# Autodesk Inventor assembly: Track Frame Assembly
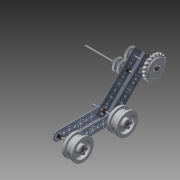
[picture p0: Inventor's stored thumbnail of the model, 180x180]
Saved by Autodesk Inventor 2015 (Build 190159000, 159)
## iProperties
Created: 2015-09-27
Part Number: Track Frame Assembly
Document SubType Name: Assembly
Designer: Jing-Chen
Author: Jing-Chen
## Documents named in this file (17)
- C:\Users\Jing-Chen\Desktop\Bionic Hybrids 2016\Bionic-Hybrids\CAD\Drivetrain\Sub-Assemblies\Track Frame Assembly.iam
- C:\Users\Jing-Chen\Desktop\Bionic Hybrids 2016\Bionic-Hybrids\Stock\Bracket-U9 - 739067.ipt
- C:\Users\Jing-Chen\Desktop\Bionic Hybrids 2016\Bionic-Hybrids\CAD\Drivetrain\Sub-Assemblies\Track Idler Assembly.iam
- C:\Users\Jing-Chen\Desktop\Bionic Hybrids 2016\Bionic-Hybrids\Stock\Bearing-Thrust - 739091.ipt
- C:\Users\Jing-Chen\Desktop\Bionic Hybrids 2016\Bionic-Hybrids\Stock\Shaft Collar-Setscrew, Axle - 739092.iam
- C:\Users\Jing-Chen\Desktop\Bionic Hybrids 2016\Bionic-Hybrids\Stock\Track Sprocket - 736468.ipt
- C:\Users\Jing-Chen\Desktop\Bionic Hybrids 2016\Bionic-Hybrids\Stock\Shaft Collar-Setscrew, Axle, Mountable - 739172.iam
- C:\Users\Jing-Chen\Desktop\Bionic Hybrids 2016\Bionic-Hybrids\Stock\Plate-9x1 - 739272.ipt
- C:\Users\Jing-Chen\Desktop\Bionic Hybrids 2016\Bionic-Hybrids\Stock\Spacer 3.125mm- 739100.ipt
- C:\Users\Jing-Chen\Desktop\Bionic Hybrids 2016\Bionic-Hybrids\Stock\Gear-40 tooth - 731901.ipt
- C:\Users\Jing-Chen\Desktop\Bionic Hybrids 2016\Bionic-Hybrids\Stock\Plate-1x1 - 739387.ipt
- C:\Users\Jing-Chen\Desktop\Bionic Hybrids 2016\Bionic-Hybrids\Stock\Screw 0.5in - 739097.ipt
- C:\Users\Jing-Chen\Desktop\Bionic Hybrids 2016\Bionic-Hybrids\CAD\General\Modified Parts\Cut 100mm axle.ipt
- C:\Users\Jing-Chen\Desktop\Bionic Hybrids 2016\Bionic-Hybrids\CAD\Drivetrain\Sub-Assemblies\Tread Sprocket Assembly.iam
- C:\Users\Jing-Chen\Desktop\Bionic Hybrids 2016\Bionic-Hybrids\Stock\Axle-250mm - 735871.ipt
- C:\Users\Jing-Chen\Desktop\Bionic Hybrids 2016\Bionic-Hybrids\CAD\General\Modified Parts\Axle Hub - non-locking.ipt
- C:\Users\Jing-Chen\Desktop\Bionic Hybrids 2016\Bionic-Hybrids\Stock\Axle-100mm - 739088.ipt
## Components (42 placed, 16 different names)
1. Bracket-U9 - 739067:1 — Mate:16, Mate:17, Mate:18, Mate:19, Mate:20, Mate:21, Mate:44, Mate:46, Mate:60, Mate:61, Mate:63, Mate:66, Mate:67, Mate:88, Mate:89, Mate:90, Mate:91, Mate:108, Mate:122, Mate:159, Mate:160, Mate:161, Mate:162, Mate:164, Mate:166, Mate:165, Mate:163
2. Track Idler Assembly:1 [sub-assembly] — Mate:43, Flush:9, Mate:134
3. Shaft Collar-Setscrew, Axle - 739092:1 [sub-assembly] — Mate:42, Mate:133
4. Track Sprocket - 736468:1 — Mate:13, Mate:15, Mate:105, Mate:126, Mate:135, Mate:136, Mate:137, Mate:138, Mate:139, Mate:140, Mate:141, Mate:142
5. Shaft Collar-Setscrew, Axle, Mountable - 739172:1 [sub-assembly] — Mate:13, Mate:15, Mate:22, Mate:105, Mate:106, Angle:3, Mate:109, Angle:5
6. Plate-9x1 - 739272:1 — Mate:16, Mate:19, Mate:21, Mate:37, Mate:38, Mate:45, Flush:4, Flush:5, Mate:53
7. Plate-9x1 - 739272:2 — Mate:17, Mate:18, Mate:20, Mate:39, Mate:40, Mate:47, Mate:179
8. Cut 100mm axle:1 — Mate:22, Mate:58, Mate:99, Mate:100, Mate:101, Angle:2, Angle:3, Mate:107, Angle:4, Mate:109, Angle:5, Mate:121, Mate:124, Mate:125, Flush:7
9. Bearing-Thrust - 739091:5 — Mate:44, Mate:45, Mate:50, Mate:175
10. Bearing-Thrust - 739091:6 — Mate:39, Mate:40, Mate:42, Mate:132
11. Bearing-Thrust - 739091:10 — Mate:46, Mate:47
12. Bearing-Thrust - 739091:11 — Mate:37, Mate:38, Mate:43
13. Track Idler Assembly:2 [sub-assembly] — Mate:50, Mate:176, Flush:10
14. Shaft Collar-Setscrew, Axle - 739092:2 [sub-assembly] — Mate:180, Mate:181
15. Gear-40 tooth - 731901:1 — Mate:55, Mate:57, Mate:64, Mate:84, Mate:85, Mate:86, Mate:87, Rotation:1
16. Shaft Collar-Setscrew, Axle, Mountable - 739172:2 [sub-assembly] — Mate:55, Mate:57, Mate:58, Mate:63, Mate:64, Angle:2, Mate:107, Mate:108, Angle:4
17. Shaft Collar-Setscrew, Axle, Mountable - 739172:4 [sub-assembly] — Mate:60, Mate:61, Mate:66, Angle:1
18. Axle-250mm - 735871:1 — Angle:1
19. Plate-1x1 - 739387:1 — Mate:67, Mate:70
20. Bearing-Thrust - 739091:12 — Mate:70, Mate:72
21. Spacer 3.125mm- 739100:3 — Mate:72, Mate:128
22. Screw 0.5in - 739097:1 — Mate:84, Mate:86
23. Screw 0.5in - 739097:2 — Mate:85, Mate:87
24. Screw 0.5in - 739097:3 — Mate:88, Mate:90
25. Screw 0.5in - 739097:4 — Mate:89, Mate:91
26. Spacer 3.125mm- 739100:5 — Mate:101, Mate:102, Mate:123, Mate:124
27. Spacer 3.125mm- 739100:6 — Mate:100, Mate:102, Mate:103
28. Spacer 3.125mm- 739100:7 — Mate:99, Mate:103, Mate:106
29. Bearing-Thrust - 739091:13 — Mate:121, Mate:122, Mate:123
30. Bearing-Thrust - 739091:14 — Mate:125, Mate:126, Flush:7
31. Tread Sprocket Assembly:1 [sub-assembly] — Mate:128, Rotation:1
32. Cut 100mm axle:3 — Flush:9, Mate:132, Mate:133, Mate:134
33. Screw 0.5in - 739097:5 — Mate:135, Mate:139
34. Screw 0.5in - 739097:6 — Mate:136, Mate:140
35. Screw 0.5in - 739097:7 — Mate:137, Mate:142
36. Screw 0.5in - 739097:8 — Mate:138, Mate:141
37. Screw 0.5in - 739097:13 — Mate:159, Mate:164, Mate:178
38. Screw 0.5in - 739097:14 — Mate:160, Mate:163
39. Screw 0.5in - 739097:15 — Mate:161, Mate:165
40. Screw 0.5in - 739097:16 — Mate:162, Mate:166
41. Axle Hub - non-locking:1 — Mate:177, Mate:178, Mate:179, Mate:181
42. Axle-100mm - 739088:1 — Mate:175, Mate:176, Flush:10, Mate:177, Mate:180
## Relationships (100: Mate 88, Flush 6, Angle 5, RelateRotation 1)
- Mate:13: Track Sprocket - 736468:1 ↔ Shaft Collar-Setscrew, Axle, Mountable - 739172:1
- Mate:15: Track Sprocket - 736468:1 ↔ Shaft Collar-Setscrew, Axle, Mountable - 739172:1
- Mate:16: Bracket-U9 - 739067:1 ↔ Plate-9x1 - 739272:1
- Mate:17: Bracket-U9 - 739067:1 ↔ Plate-9x1 - 739272:2
- Mate:18: Bracket-U9 - 739067:1 ↔ Plate-9x1 - 739272:2
- Mate:19: Bracket-U9 - 739067:1 ↔ Plate-9x1 - 739272:1
- Mate:20: Bracket-U9 - 739067:1 ↔ Plate-9x1 - 739272:2
- Mate:21: Bracket-U9 - 739067:1 ↔ Plate-9x1 - 739272:1
- Mate:22: Shaft Collar-Setscrew, Axle, Mountable - 739172:1 ↔ Cut 100mm axle:1
- Mate:37: Plate-9x1 - 739272:1 ↔ Bearing-Thrust - 739091:11
- Mate:38: Plate-9x1 - 739272:1 ↔ Bearing-Thrust - 739091:11
- Mate:39: Plate-9x1 - 739272:2 ↔ Bearing-Thrust - 739091:6
- Mate:40: Plate-9x1 - 739272:2 ↔ Bearing-Thrust - 739091:6
- Mate:42: Shaft Collar-Setscrew, Axle - 739092:1 ↔ Bearing-Thrust - 739091:6
- Mate:43: Track Idler Assembly:1 ↔ Bearing-Thrust - 739091:11
- Mate:44: Bracket-U9 - 739067:1 ↔ Bearing-Thrust - 739091:5
- Mate:45: Plate-9x1 - 739272:1 ↔ Bearing-Thrust - 739091:5
- Mate:46: Bracket-U9 - 739067:1 ↔ Bearing-Thrust - 739091:10
- Mate:47: Plate-9x1 - 739272:2 ↔ Bearing-Thrust - 739091:10
- Mate:50: Bearing-Thrust - 739091:5 ↔ Track Idler Assembly:2
- Flush:4: Plate-9x1 - 739272:1
- Flush:5: Plate-9x1 - 739272:1
- Mate:53: Plate-9x1 - 739272:1
- Mate:55: Gear-40 tooth - 731901:1 ↔ Shaft Collar-Setscrew, Axle, Mountable - 739172:2
- Mate:57: Gear-40 tooth - 731901:1 ↔ Shaft Collar-Setscrew, Axle, Mountable - 739172:2
- Mate:58: Cut 100mm axle:1 ↔ Shaft Collar-Setscrew, Axle, Mountable - 739172:2
- Mate:60: Bracket-U9 - 739067:1 ↔ Shaft Collar-Setscrew, Axle, Mountable - 739172:4
- Mate:61: Bracket-U9 - 739067:1 ↔ Shaft Collar-Setscrew, Axle, Mountable - 739172:4
- Mate:63: Bracket-U9 - 739067:1 ↔ Shaft Collar-Setscrew, Axle, Mountable - 739172:2
- Mate:64: Gear-40 tooth - 731901:1 ↔ Shaft Collar-Setscrew, Axle, Mountable - 739172:2
- [Mate]: Shaft Collar-Setscrew, Axle, Mountable - 739172:4 ↔ Axle-250mm - 735871:1
- [Flush]: Shaft Collar-Setscrew, Axle, Mountable - 739172:4 ↔ Axle-250mm - 735871:1
- Mate:66: Bracket-U9 - 739067:1 ↔ Shaft Collar-Setscrew, Axle, Mountable - 739172:4
- Mate:67: Bracket-U9 - 739067:1 ↔ Plate-1x1 - 739387:1
- [Mate]: Axle-250mm - 735871:1 ↔ Plate-1x1 - 739387:1
- [Mate]: Axle-250mm - 735871:1 ↔ Bearing-Thrust - 739091:12
- Mate:70: Plate-1x1 - 739387:1 ↔ Bearing-Thrust - 739091:12
- [Mate]: Axle-250mm - 735871:1 ↔ Spacer 3.125mm- 739100:3
- Mate:72: Bearing-Thrust - 739091:12 ↔ Spacer 3.125mm- 739100:3
- Angle:1 (180 deg): Shaft Collar-Setscrew, Axle, Mountable - 739172:4 ↔ Axle-250mm - 735871:1
- Mate:84: Gear-40 tooth - 731901:1 ↔ Screw 0.5in - 739097:1
- Mate:85: Gear-40 tooth - 731901:1 ↔ Screw 0.5in - 739097:2
- Mate:86: Gear-40 tooth - 731901:1 ↔ Screw 0.5in - 739097:1
- Mate:87: Gear-40 tooth - 731901:1 ↔ Screw 0.5in - 739097:2
- Mate:88: Bracket-U9 - 739067:1 ↔ Screw 0.5in - 739097:3
- Mate:89: Bracket-U9 - 739067:1 ↔ Screw 0.5in - 739097:4
- Mate:90: Bracket-U9 - 739067:1 ↔ Screw 0.5in - 739097:3
- Mate:91: Bracket-U9 - 739067:1 ↔ Screw 0.5in - 739097:4
- Mate:99: Cut 100mm axle:1 ↔ Spacer 3.125mm- 739100:7
- Mate:100: Cut 100mm axle:1 ↔ Spacer 3.125mm- 739100:6
- Mate:101: Cut 100mm axle:1 ↔ Spacer 3.125mm- 739100:5
- Mate:102: Spacer 3.125mm- 739100:5 ↔ Spacer 3.125mm- 739100:6
- Mate:103: Spacer 3.125mm- 739100:6 ↔ Spacer 3.125mm- 739100:7
- Mate:105: Track Sprocket - 736468:1 ↔ Shaft Collar-Setscrew, Axle, Mountable - 739172:1
- Mate:106: Shaft Collar-Setscrew, Axle, Mountable - 739172:1 ↔ Spacer 3.125mm- 739100:7
- Angle:2 (180 deg): Cut 100mm axle:1 ↔ Shaft Collar-Setscrew, Axle, Mountable - 739172:2
- Angle:3 (180 deg): Shaft Collar-Setscrew, Axle, Mountable - 739172:1 ↔ Cut 100mm axle:1
- Mate:107: Cut 100mm axle:1 ↔ Shaft Collar-Setscrew, Axle, Mountable - 739172:2
- Mate:108: Bracket-U9 - 739067:1 ↔ Shaft Collar-Setscrew, Axle, Mountable - 739172:2
- Angle:4 (180 deg): Cut 100mm axle:1 ↔ Shaft Collar-Setscrew, Axle, Mountable - 739172:2
- Mate:109: Shaft Collar-Setscrew, Axle, Mountable - 739172:1 ↔ Cut 100mm axle:1
- Angle:5 (180 deg): Shaft Collar-Setscrew, Axle, Mountable - 739172:1 ↔ Cut 100mm axle:1
- Mate:121: Cut 100mm axle:1 ↔ Bearing-Thrust - 739091:13
- Mate:122: Bracket-U9 - 739067:1 ↔ Bearing-Thrust - 739091:13
- Mate:123: Spacer 3.125mm- 739100:5 ↔ Bearing-Thrust - 739091:13
- Mate:124: Cut 100mm axle:1 ↔ Spacer 3.125mm- 739100:5
- Mate:125: Cut 100mm axle:1 ↔ Bearing-Thrust - 739091:14
- Mate:126: Track Sprocket - 736468:1 ↔ Bearing-Thrust - 739091:14
- Flush:7: Cut 100mm axle:1 ↔ Bearing-Thrust - 739091:14
- [Mate]: Axle-250mm - 735871:1 ↔ Tread Sprocket Assembly:1
- Mate:128: Spacer 3.125mm- 739100:3 ↔ Tread Sprocket Assembly:1
- Rotation:1 [RelateRotation] (1 ul): Gear-40 tooth - 731901:1 ↔ Tread Sprocket Assembly:1
- Flush:9: Track Idler Assembly:1 ↔ Cut 100mm axle:3
- Mate:132: Bearing-Thrust - 739091:6 ↔ Cut 100mm axle:3
- Mate:133: Shaft Collar-Setscrew, Axle - 739092:1 ↔ Cut 100mm axle:3
- Mate:134: Track Idler Assembly:1 ↔ Cut 100mm axle:3
- Mate:135: Track Sprocket - 736468:1 ↔ Screw 0.5in - 739097:5
- Mate:136: Track Sprocket - 736468:1 ↔ Screw 0.5in - 739097:6
- Mate:137: Track Sprocket - 736468:1 ↔ Screw 0.5in - 739097:7
- Mate:138: Track Sprocket - 736468:1 ↔ Screw 0.5in - 739097:8
- Mate:139: Track Sprocket - 736468:1 ↔ Screw 0.5in - 739097:5
- Mate:140: Track Sprocket - 736468:1 ↔ Screw 0.5in - 739097:6
- Mate:141: Track Sprocket - 736468:1 ↔ Screw 0.5in - 739097:8
- Mate:142: Track Sprocket - 736468:1 ↔ Screw 0.5in - 739097:7
- Mate:159: Bracket-U9 - 739067:1 ↔ Screw 0.5in - 739097:13
- Mate:160: Bracket-U9 - 739067:1 ↔ Screw 0.5in - 739097:14
- Mate:161: Bracket-U9 - 739067:1 ↔ Screw 0.5in - 739097:15
- Mate:162: Bracket-U9 - 739067:1 ↔ Screw 0.5in - 739097:16
- Mate:163: Bracket-U9 - 739067:1 ↔ Screw 0.5in - 739097:14
- Mate:164: Bracket-U9 - 739067:1 ↔ Screw 0.5in - 739097:13
- Mate:165: Bracket-U9 - 739067:1 ↔ Screw 0.5in - 739097:15
- Mate:166: Bracket-U9 - 739067:1 ↔ Screw 0.5in - 739097:16
- Mate:175: Bearing-Thrust - 739091:5 ↔ Axle-100mm - 739088:1
- Mate:176: Track Idler Assembly:2 ↔ Axle-100mm - 739088:1
- Flush:10: Track Idler Assembly:2 ↔ Axle-100mm - 739088:1
- Mate:177: Axle Hub - non-locking:1 ↔ Axle-100mm - 739088:1
- Mate:178: Screw 0.5in - 739097:13 ↔ Axle Hub - non-locking:1
- Mate:179: Plate-9x1 - 739272:2 ↔ Axle Hub - non-locking:1
- Mate:180: Shaft Collar-Setscrew, Axle - 739092:2 ↔ Axle-100mm - 739088:1
- Mate:181: Shaft Collar-Setscrew, Axle - 739092:2 ↔ Axle Hub - non-locking:1
